# Autodesk Inventor assembly: electrical board front
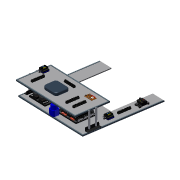
[picture p0: Inventor's stored thumbnail of the model, 180x180]
Saved by Autodesk Inventor 2012 (Build 160160000, 160)
## iProperties
Created: 2012-01-14
Part Number: electrical board front
Document SubType Name: Assembly
Designer: Antonella Wilby
Author: Antonella Wilby
## Documents named in this file (12)
- C:\Users\Antonella\Documents\GCC Robotics 2012 - Mechanical\Robot 2.0\Electrical\Front Electrical Board\Front Electrical Board.iam
- C:\Users\Antonella\Documents\GCC Robotics 2012 - Mechanical\Robot 2.0\Electrical\Front Electrical Board\Bottom\Electrical Board - front bottom.iam
- C:\Users\Antonella\Documents\GCC Robotics 2012 - Mechanical\Robot 2.0\Electrical\Front Electrical Board\Top\Electrical Board - front top.iam
- C:\Users\Antonella\Documents\GCC Robotics 2012 - Mechanical\Robot 2.0\Electrical\Front Electrical Board\top bottom link.ipt
- C:\Users\Antonella\Documents\GCC Robotics 2012 - Mechanical\Robot 2.0\Other Models\DirectMountTerminalBlock_AutomationDirect_BM-M092CS.iam
- C:\Users\Antonella\Documents\GCC Robotics 2012 - Mechanical\Robot 2.0\Other Models\Circuit Breaker\CircuitBreaker_TSC_CB3-SM-120.iam
- C:\Users\Antonella\Documents\GCC Robotics 2012 - Mechanical\Robot 2.0\Other Models\Operator Interface\Operator Interface.iam
- C:\Users\Antonella\Documents\GCC Robotics 2012 - Mechanical\Robot 2.0\Electrical\URG\rangefinder model.ipt
- C:\Users\Antonella\Documents\GCC Robotics 2012 - Mechanical\Robot 2.0\Other Models\Breaker Panel\Breaker Panel.iam
- C:\Users\Antonella\Documents\GCC Robotics 2012 - Mechanical\Robot 2.0\Other Models\IR Board\2008 IR Board.iam
- C:\Users\Antonella\Documents\GCC Robotics 2012 - Mechanical\Robot 2.0\Other Models\Relay\Spike H.iam
- C:\Users\Antonella\Documents\GCC Robotics 2012 - Mechanical\Robot 2.0\Other Models\router.ipt
## Components (19 placed, 11 different names)
1. Electrical Board - front bottom:1 [sub-assembly] — Mate:1, Mate:3, Mate:4, Mate:5, Mate:6, Mate:7, Mate:8, Mate:9, Mate:10, Mate:20, Flush:5, Mate:21, Flush:6, Mate:22, Flush:7, Mate:23, Flush:8, Mate:24, Flush:9, Mate:26, Mate:27
2. Electrical Board - front top:1 [sub-assembly] — Mate:1, Mate:11, Mate:12, Mate:13, Mate:14, Mate:15, Flush:1, Mate:16, Flush:2, Mate:17, Mate:19, Flush:4, Mate:25, Flush:10, Mate:28, Mate:29, Flush:11, Flush:12, Mate:30, Mate:31, Flush:14
3. top bottom link:1 — Mate:5, Mate:6, Mate:12
4. top bottom link:2 — Mate:3, Mate:4, Mate:11
5. top bottom link:3 — Mate:7, Mate:8, Mate:13
6. top bottom link:4 — Mate:9, Mate:10, Mate:14
7. DirectMountTerminalBlock_AutomationDirect_BM-M092CS:1 [sub-assembly] — Mate:15, Flush:1, Flush:13
8. DirectMountTerminalBlock_AutomationDirect_BM-M092CS:2 [sub-assembly] — Mate:19, Flush:4
9. DirectMountTerminalBlock_AutomationDirect_BM-M092CS:3 [sub-assembly] — Mate:17, Mate:18, Flush:3, Flush:13
10. DirectMountTerminalBlock_AutomationDirect_BM-M092CS:4 [sub-assembly] — Mate:16, Flush:2, Mate:18, Flush:3, Flush:12
11. CircuitBreaker_TSC_CB3-SM-120:1 [sub-assembly] — Mate:20, Flush:5
12. DirectMountTerminalBlock_AutomationDirect_BM-M092CS:5 [sub-assembly] — Mate:21, Flush:6
13. Operator Interface:1 [sub-assembly] — Mate:22, Flush:7
14. rangefinder model:1 — Mate:23, Flush:8
15. Breaker Panel:1 [sub-assembly] — Mate:24, Flush:9
16. 2008 IR Board:1 [sub-assembly] — Mate:25, Flush:10, Flush:11
17. Spike H:1 [sub-assembly] — Mate:26, Mate:27
18. Spike H:2 [sub-assembly] — Mate:28, Mate:29, Mate:30
19. router:1 — Mate:31, Flush:14
## Relationships (44: Mate 30, Flush 14)
- Mate:1: Electrical Board - front bottom:1 ↔ Electrical Board - front top:1
- Mate:3: Electrical Board - front bottom:1 ↔ top bottom link:2
- Mate:4: Electrical Board - front bottom:1 ↔ top bottom link:2
- Mate:5: Electrical Board - front bottom:1 ↔ top bottom link:1
- Mate:6: Electrical Board - front bottom:1 ↔ top bottom link:1
- Mate:7: Electrical Board - front bottom:1 ↔ top bottom link:3
- Mate:8: Electrical Board - front bottom:1 ↔ top bottom link:3
- Mate:9: Electrical Board - front bottom:1 ↔ top bottom link:4
- Mate:10: Electrical Board - front bottom:1 ↔ top bottom link:4
- Mate:11: Electrical Board - front top:1 ↔ top bottom link:2
- Mate:12: Electrical Board - front top:1 ↔ top bottom link:1
- Mate:13: Electrical Board - front top:1 ↔ top bottom link:3
- Mate:14: Electrical Board - front top:1 ↔ top bottom link:4
- Mate:15: Electrical Board - front top:1 ↔ DirectMountTerminalBlock_AutomationDirect_BM-M092CS:1
- Flush:1 (-76.2 mm): Electrical Board - front top:1 ↔ DirectMountTerminalBlock_AutomationDirect_BM-M092CS:1
- Mate:16: Electrical Board - front top:1 ↔ DirectMountTerminalBlock_AutomationDirect_BM-M092CS:4
- Flush:2 (-76.2 mm): Electrical Board - front top:1 ↔ DirectMountTerminalBlock_AutomationDirect_BM-M092CS:4
- Mate:17: Electrical Board - front top:1 ↔ DirectMountTerminalBlock_AutomationDirect_BM-M092CS:3
- Mate:18 (50.8 mm): DirectMountTerminalBlock_AutomationDirect_BM-M092CS:3 ↔ DirectMountTerminalBlock_AutomationDirect_BM-M092CS:4
- Flush:3: DirectMountTerminalBlock_AutomationDirect_BM-M092CS:3 ↔ DirectMountTerminalBlock_AutomationDirect_BM-M092CS:4
- Mate:19: Electrical Board - front top:1 ↔ DirectMountTerminalBlock_AutomationDirect_BM-M092CS:2
- Flush:4 (-50.8 mm): Electrical Board - front top:1 ↔ DirectMountTerminalBlock_AutomationDirect_BM-M092CS:2
- Mate:20: Electrical Board - front bottom:1 ↔ CircuitBreaker_TSC_CB3-SM-120:1
- Flush:5 (25.4 mm): Electrical Board - front bottom:1 ↔ CircuitBreaker_TSC_CB3-SM-120:1
- Mate:21: Electrical Board - front bottom:1 ↔ DirectMountTerminalBlock_AutomationDirect_BM-M092CS:5
- Flush:6 (50.8 mm): Electrical Board - front bottom:1 ↔ DirectMountTerminalBlock_AutomationDirect_BM-M092CS:5
- Mate:22: Electrical Board - front bottom:1 ↔ Operator Interface:1
- Flush:7 (50.8 mm): Electrical Board - front bottom:1 ↔ Operator Interface:1
- Mate:23: Electrical Board - front bottom:1 ↔ rangefinder model:1
- Flush:8: Electrical Board - front bottom:1 ↔ rangefinder model:1
- Mate:24: Electrical Board - front bottom:1 ↔ Breaker Panel:1
- Flush:9 (38.1 mm): Electrical Board - front bottom:1 ↔ Breaker Panel:1
- Mate:25: Electrical Board - front top:1 ↔ 2008 IR Board:1
- Flush:10 (-76.2 mm): Electrical Board - front top:1 ↔ 2008 IR Board:1
- Mate:26: Electrical Board - front bottom:1 ↔ Spike H:1
- Mate:27 (-38.1 mm): Electrical Board - front bottom:1 ↔ Spike H:1
- Mate:28: Electrical Board - front top:1 ↔ Spike H:2
- Mate:29 (-50.8 mm): Electrical Board - front top:1 ↔ Spike H:2
- Flush:11 (-38.1 mm): Electrical Board - front top:1 ↔ 2008 IR Board:1
- Flush:12 (50.8 mm): Electrical Board - front top:1 ↔ DirectMountTerminalBlock_AutomationDirect_BM-M092CS:4
- Flush:13: DirectMountTerminalBlock_AutomationDirect_BM-M092CS:1 ↔ DirectMountTerminalBlock_AutomationDirect_BM-M092CS:3
- Mate:30 (-50.8 mm): Electrical Board - front top:1 ↔ Spike H:2
- Mate:31: Electrical Board - front top:1 ↔ router:1
- Flush:14 (50.8 mm): Electrical Board - front top:1 ↔ router:1
